# Autodesk Inventor assembly: ASY GBK 2330 short wall shield 9
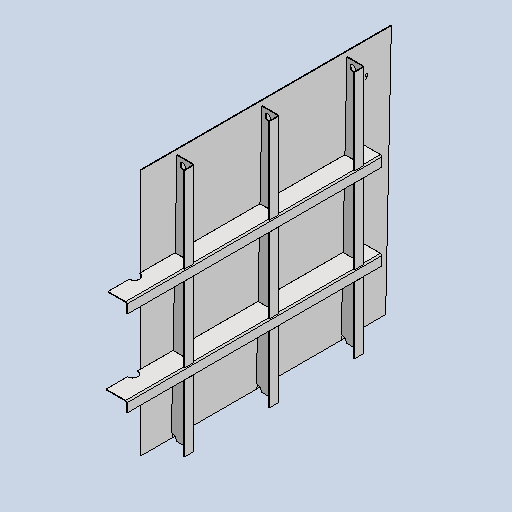
[picture p0: Inventor's stored thumbnail of the model, 512x512]
Saved by Autodesk Inventor 2026.2 (Build 302298010, 298A)
## iProperties
Created: 2026-05-07
Part Number: ASY GBK 2330 short wall shield 9
Document SubType Name: Assembly
Designer: pokla
Mass: 107756 g
Surface Area: 69611.7 cm^2
Volume: 13726.9 cm^3
Density: 7.85 g/cm^3
Author: admin
## Documents named in this file (6)
- C:\Users\admin\Documents\Inventor\GBK-Gubkinskiy\ASY GBK 2330 short wall shield 9.iam
- C:\Users\admin\Documents\Inventor\GBK-Gubkinskiy\GBK 0101 main rib.ipt
- C:\Users\admin\Documents\Inventor\GBK-Gubkinskiy\GBK 2331 shield 9.ipt
- C:\Users\admin\Documents\Inventor\GBK-Gubkinskiy\GBK 0302 stringer 7.ipt
- C:\Users\admin\Documents\Inventor\GBK-Gubkinskiy\GBK 0303 stringer 8.ipt
- C:\Users\admin\Documents\Inventor\GBK-Gubkinskiy\GBK 0301 third rib.ipt
## Components (6 placed, 4 different names)
1. GBK 0302 stringer 7.ipt:1 — Rigid:1
2. GBK 0303 stringer 8.ipt:1 — Rigid:2, Flush:4
3. GBK 2331 shield 9.ipt:1 — Mate:1, Mate:2, Flush:4, Mate:4
4. GBK 0301 third rib.ipt:1 — Mate:1, Mate:2, Rigid:2, Rigid:1, Mate:3, Flush:5
5. GBK 0301 third rib.ipt:2
6. GBK 0301 third rib.ipt:3
## Component patterns: (3 elements, first: GBK 0301 third rib.ipt:1)
## Relationships (8: Mate 4, WeldJoint 2, Flush 2)
- Mate:1: GBK 2331 shield 9.ipt:1 ↔ GBK 0301 third rib.ipt:1
- Mate:2: GBK 2331 shield 9.ipt:1 ↔ GBK 0301 third rib.ipt:1
- Rigid:2 [WeldJoint] (4 mm): GBK 0303 stringer 8.ipt:1 ↔ GBK 0301 third rib.ipt:1
- Rigid:1 [WeldJoint] (4 mm): GBK 0302 stringer 7.ipt:1 ↔ GBK 0301 third rib.ipt:1
- Flush:4 (155 mm): GBK 0303 stringer 8.ipt:1 ↔ GBK 2331 shield 9.ipt:1
- Mate:3: GBK 0301 third rib.ipt:1
- Mate:4: GBK 2331 shield 9.ipt:1
- Flush:5: GBK 0301 third rib.ipt:1
## Named parameters: основание_длина_нижнего = 200 mm, основание_длина_верхнего = 100 mm, стрингер_глубина_1 = 190.70056 mm, стрингер_глубина_2 = 179.35977 mm, стрингер_глубина_3 = 168.01899 mm, стрингер_глубина_4 = 156.6782 mm, стрингер_глубина_5 = 145.33742 mm, стрингер_глубина_6 = 133.99663 mm, стрингер_глубина_7 = 122.65585 mm, стрингер_глубина_8 = 111.31507 mm, Лист_ширина = 1480 mm, ребро_усилителей = 60 mm, паз_под_стрингер_глубина = 70 mm, паз_под_стрингер_толщина = 5 mm, отступ_от_пола_до_первого_стрингера = 410 mm, шаг_стрингеров = 500 mm, радиус_выреза_под_сварку = 30 mm, нахлест_шпангоутов_1_2 = 150 mm, нахлест_шпангоутов_2_3 = 120 mm, Стрингер_длина = 1489.5 mm, Лист_длина = 2980 mm, Шаг_шпангоутов = 496.66667 mm
